# Autodesk Inventor assembly: EnsembleServoTobogan
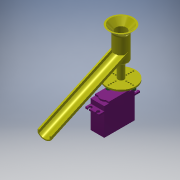
[picture p0: Inventor's stored thumbnail of the model, 180x180]
Saved by Autodesk Inventor 2019 (Build 230136000, 136)
## iProperties
Created: 2021-01-22
Part Number: EnsembleServoTobogan
Material: Générique
Document SubType Name: Assembly
Designer: tom.mousset
Author: tom.mousset
## Documents named in this file (4)
- D:\triSmarties\EnsembleServoTobogan.iam
- D:\erasmus\moteur.ipt
- D:\triSmarties\palonnierServo.ipt
- D:\triSmarties\toboganANavet.ipt
## Components (3 placed, 3 different names)
1. moteur:1 — Placage:1, Placage:2
2. palonnierServo:1 — Placage:1, Placage:2, Placage:3, Placage:4, Angle:1
3. toboganANavet:1 — Placage:3, Placage:4, Angle:1
## Relationships (5: Mate 4, Angle 1)
- Placage:1 [Mate]: moteur:1 ↔ palonnierServo:1
- Placage:2 [Mate] (6 mm): moteur:1 ↔ palonnierServo:1
- Placage:3 [Mate]: palonnierServo:1 ↔ toboganANavet:1
- Placage:4 [Mate]: palonnierServo:1 ↔ toboganANavet:1
- Angle:1 (0 deg): palonnierServo:1 ↔ toboganANavet:1
